# Autodesk Inventor assembly: motor_krilo
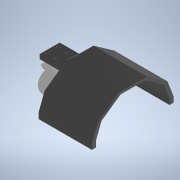
[picture p0: Inventor's stored thumbnail of the model, 180x180]
Saved by Autodesk Inventor 2022 (Build 260153000, 153)
## iProperties
Created: 2023-05-18
Part Number: motor_krilo
Document SubType Name: Assembly
Designer: Robo0
Author: Robo0
## Documents named in this file (4)
- C:\git\robot_01\design\motor_krilo.iam
- C:\git\robot_01\design\mot137.ipt
- C:\git\robot_01\design\krilo.ipt
- C:\git\robot_01\design\Двигатель.ipt
## Components (3 placed, 3 different names)
1. mot137:1 — Совмещение:1, Совмещение:2, Совмещение:3, Совмещение:4, Совмещение:5, Совмещение:6
2. krilo:1 — Совмещение:1, Совмещение:2, Совмещение:3
3. Двигатель:1 — Совмещение:4, Совмещение:5, Совмещение:6
## Relationships (6: Mate 6)
- Совмещение:1 [Mate]: mot137:1 ↔ krilo:1
- Совмещение:2 [Mate]: mot137:1 ↔ krilo:1
- Совмещение:3 [Mate] (6 mm): mot137:1 ↔ krilo:1
- Совмещение:4 [Mate]: mot137:1 ↔ Двигатель:1
- Совмещение:5 [Mate]: mot137:1 ↔ Двигатель:1
- Совмещение:6 [Mate]: mot137:1 ↔ Двигатель:1
